# Autodesk Inventor assembly: Узел емкости
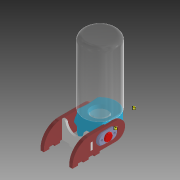
[picture p0: Inventor's stored thumbnail of the model, 180x180]
Saved by Autodesk Inventor 2022 (Build 260153000, 153)
## iProperties
Created: 2025-01-23
Part Number: Узел емкости
Document SubType Name: Assembly
Designer: Ivan
Mass: 11718.9 g
Surface Area: 16232.6 cm^2
Volume: 11718.9 cm^3
Density: 1 g/cm^3
Author: Ivan
Title: Узел емкости
## Documents named in this file (14)
- E:\Предпроф 2025\Shoter_1_ZIP\Узел емкости.iam
- E:\Предпроф 2025\Shoter_1_ZIP\Основание.ipt
- E:\Предпроф 2025\Shoter_1_ZIP\Палец.ipt
- E:\Предпроф 2025\Shoter_1_ZIP\Крышка пальца.ipt
- E:\Предпроф 2025\Shoter_1_ZIP\Стенка.ipt
- E:\Предпроф 2025\Shoter_1_ZIP\Фанера_1.ipt
- E:\Предпроф 2025\Shoter_1_ZIP\Фанера_2.ipt
- E:\Предпроф 2025\Shoter_1_ZIP\Фанера_3.ipt
- E:\Предпроф 2025\Shoter_1_ZIP\Фанера_4.ipt
- E:\Предпроф 2025\Shoter_1_ZIP\Фанера_5.ipt
- E:\Предпроф 2025\Shoter_1_ZIP\Фанера_6.ipt
- E:\Предпроф 2025\Shoter_1_ZIP\Бутылка.ipt
- E:\Предпроф 2025\Shoter_1_ZIP\Основание кнопки.ipt
- E:\Предпроф 2025\Shoter_1_ZIP\Кнопка.ipt
## Components (13 placed, 13 different names)
1. Основание:1 — Совмещение:1, Заподлицо:1, Совмещение:2, Совмещение:3, Совмещение:4, Заподлицо:4, Совмещение:11, Заподлицо:7, Совмещение:12, Совмещение:17, Совмещение:18
2. Палец:1 — Совмещение:2, Заподлицо:2
3. Крышка пальца:1 — Совмещение:1, Заподлицо:1, Заподлицо:2
4. Стенка:1 — Заподлицо:6, Совмещение:9, Совмещение:10
5. Фанера_1:1 — Совмещение:3, Совмещение:4, Совмещение:5, Совмещение:6, Заподлицо:3, Заподлицо:4, Совмещение:9, Совмещение:10
6. Фанера_2:1 — Совмещение:5, Совмещение:6, Заподлицо:3, Совмещение:7, Заподлицо:5, Совмещение:8
7. Фанера_3:1 — Совмещение:7, Заподлицо:5, Совмещение:8, Заподлицо:6, Совмещение:19, Совмещение:20, Совмещение:21
8. Фанера_4:1 — Совмещение:11, Заподлицо:7, Совмещение:12, Совмещение:13, Заподлицо:8, Совмещение:14
9. Фанера_5:1 — Совмещение:13, Заподлицо:8, Совмещение:14, Совмещение:15, Совмещение:16, Заподлицо:9
10. Фанера_6:1 — Совмещение:15, Совмещение:16, Заподлицо:9
11. Бутылка:1 — Совмещение:17, Совмещение:18
12. Основание кнопки:1 — Совмещение:19, Совмещение:20, Совмещение:21, Совмещение:22, Заподлицо:10
13. Кнопка:1 — Совмещение:22, Заподлицо:10
## Relationships (32: Mate 22, Flush 10)
- Совмещение:1 [Mate]: Основание:1 ↔ Крышка пальца:1
- Заподлицо:1 [Flush]: Основание:1 ↔ Крышка пальца:1
- Совмещение:2 [Mate]: Основание:1 ↔ Палец:1
- Заподлицо:2 [Flush] (-6 mm): Палец:1 ↔ Крышка пальца:1
- Совмещение:3 [Mate]: Основание:1 ↔ Фанера_1:1
- Совмещение:4 [Mate]: Основание:1 ↔ Фанера_1:1
- Совмещение:5 [Mate]: Фанера_1:1 ↔ Фанера_2:1
- Совмещение:6 [Mate]: Фанера_1:1 ↔ Фанера_2:1
- Заподлицо:3 [Flush]: Фанера_1:1 ↔ Фанера_2:1
- Заподлицо:4 [Flush]: Основание:1 ↔ Фанера_1:1
- Совмещение:7 [Mate]: Фанера_2:1 ↔ Фанера_3:1
- Заподлицо:5 [Flush]: Фанера_2:1 ↔ Фанера_3:1
- Совмещение:8 [Mate]: Фанера_2:1 ↔ Фанера_3:1
- Заподлицо:6 [Flush]: Стенка:1 ↔ Фанера_3:1
- Совмещение:9 [Mate]: Стенка:1 ↔ Фанера_1:1
- Совмещение:10 [Mate]: Стенка:1 ↔ Фанера_1:1
- Совмещение:11 [Mate]: Основание:1 ↔ Фанера_4:1
- Заподлицо:7 [Flush]: Основание:1 ↔ Фанера_4:1
- Совмещение:12 [Mate]: Основание:1 ↔ Фанера_4:1
- Совмещение:13 [Mate]: Фанера_4:1 ↔ Фанера_5:1
- Заподлицо:8 [Flush]: Фанера_4:1 ↔ Фанера_5:1
- Совмещение:14 [Mate]: Фанера_4:1 ↔ Фанера_5:1
- Совмещение:15 [Mate]: Фанера_5:1 ↔ Фанера_6:1
- Совмещение:16 [Mate]: Фанера_5:1 ↔ Фанера_6:1
- Заподлицо:9 [Flush]: Фанера_5:1 ↔ Фанера_6:1
- Совмещение:17 [Mate]: Основание:1 ↔ Бутылка:1
- Совмещение:18 [Mate]: Основание:1 ↔ Бутылка:1
- Совмещение:19 [Mate]: Фанера_3:1 ↔ Основание кнопки:1
- Совмещение:20 [Mate]: Фанера_3:1 ↔ Основание кнопки:1
- Совмещение:21 [Mate]: Фанера_3:1 ↔ Основание кнопки:1
- Совмещение:22 [Mate]: Основание кнопки:1 ↔ Кнопка:1
- Заподлицо:10 [Flush] (-3 mm): Основание кнопки:1 ↔ Кнопка:1
